# Autodesk Inventor assembly: 50cal_truck
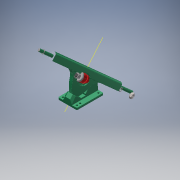
[picture p0: Inventor's stored thumbnail of the model, 180x180]
Saved by Autodesk Inventor 2018 (Build 220112000, 112)
## iProperties
Created: 2014-01-03
Part Number: 50cal_truck
Document SubType Name: Assembly
Designer: Rus
Sending System: SolidWorks 2014
Last Author: mcooper
Last Saved: 2015-06-04
Author: Rus
## Documents named in this file (12)
- C:\Users\Rus\Documents\3D Models\Electric Longboard\Trucks\50_CAL\50cal_truck.iam
- C:\Users\Rus\Documents\3D Models\Electric Longboard\Trucks\50_CAL\50cal_baseplate.ipt
- C:\Users\Rus\Documents\3D Models\Electric Longboard\Trucks\50_CAL\10cal_hanger.ipt
- C:\Users\Rus\Documents\3D Models\Electric Longboard\Trucks\50_CAL\BS_bushing.ipt
- C:\Users\Rus\Documents\3D Models\Electric Longboard\Trucks\50_CAL\BS_washer.ipt
- C:\Users\Rus\Documents\3D Models\Electric Longboard\Trucks\50_CAL\kingpin.ipt
- C:\Users\Rus\Documents\3D Models\Electric Longboard\Trucks\50_CAL\Pivot_cup.ipt
- C:\Users\Rus\Documents\3D Models\Electric Longboard\Trucks\50_CAL\RS_bushing.ipt
- C:\Users\Rus\Documents\3D Models\Electric Longboard\Trucks\50_CAL\RS_washer.ipt
- C:\Users\Rus\Documents\3D Models\Electric Longboard\Trucks\50_CAL\kingpin-nut.ipt
- C:\Users\Rus\Documents\3D Models\Electric Longboard\Trucks\50_CAL\washer.ipt
- C:\Users\Rus\Documents\3D Models\Electric Longboard\Trucks\50_CAL\Axle-nut.ipt
## Components (12 placed, 11 different names)
1. 50cal_baseplate:1 — Insert:1, Mate:4, Angle:1, Insert:2, Insert:4
2. 10cal_hanger:1 — Mate:5, Tangent:1, Angle:2
3. BS_bushing:1 — Mate:7, Insert:3
4. BS_washer:1 — Mate:7, Insert:3, Insert:4
5. kingpin:1 — Insert:1, Mate:1, Mate:2, Mate:3
6. Pivot_cup:1 — Mate:6, Tangent:1, Insert:2, Angle:2
7. RS_bushing:1
8. RS_washer:1
9. kingpin-nut:1
10. washer:1
11. washer:5
12. Axle-nut:1
## Relationships (15: Mate 7, Insert 4, Angle 2, Flush 1, Tangent 1)
- Insert:1: 50cal_baseplate:1 ↔ kingpin:1
- Mate:1: kingpin:1
- Mate:2: kingpin:1
- Mate:3: kingpin:1
- Mate:4: 50cal_baseplate:1
- Angle:1 (0 deg): 50cal_baseplate:1
- Flush:1
- Mate:5: 10cal_hanger:1
- Mate:6: Pivot_cup:1
- Tangent:1: 10cal_hanger:1 ↔ Pivot_cup:1
- Insert:2: 50cal_baseplate:1 ↔ Pivot_cup:1
- Angle:2 (0 deg): 10cal_hanger:1 ↔ Pivot_cup:1
- Mate:7: BS_bushing:1 ↔ BS_washer:1
- Insert:3: BS_bushing:1 ↔ BS_washer:1
- Insert:4: 50cal_baseplate:1 ↔ BS_washer:1
